# Autodesk Inventor assembly: manifold
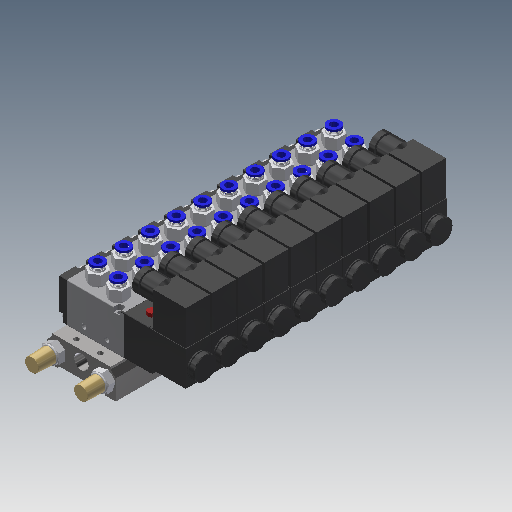
[picture p0: Inventor's stored thumbnail of the model, 512x512]
Saved by Autodesk Inventor 2017 (Build 210142000, 142)
## iProperties
Created: 2018-06-21
Part Number: manifold
Document SubType Name: Assembly
Designer: Luiz Gustavo
Author: Luiz Gustavo
## Documents named in this file (5)
- C:\Users\Luiz Gustavo\Documents\Inventor\piano-robot\manifold.iam
- C:\Users\Luiz Gustavo\Documents\Inventor\piano-robot\manifold-block.ipt
- C:\Users\Luiz Gustavo\Documents\Inventor\piano-robot\grabcad\AIRTAC 4V21008\4V21008.ipt
- C:\Users\Luiz Gustavo\Documents\Inventor\piano-robot\grabcad\AIRTAC 4V21008\BSL02.ipt
- C:\Users\Luiz Gustavo\Documents\Inventor\piano-robot\grabcad\AIRTAC 4V21008\PC602.ipt
## Components (35 placed, 4 different names)
1. manifold-block:1 — Flush:1, Flush:2, Flush:3, Rigid:1, Rigid:2, Rigid:3, Rigid:4, Rigid:5
2. BSL02:1 — Rigid:2
3. BSL02:2 — Rigid:3
4. BSL02:3 — Rigid:5
5. BSL02:4 — Rigid:4
6. 4V21008:1 — Rigid:1, Rigid:6, Rigid:7
7. 4V21008:2
8. 4V21008:3
9. 4V21008:4
10. 4V21008:5
11. 4V21008:6
12. 4V21008:7
13. 4V21008:8
14. 4V21008:9
15. 4V21008:10
16. PC602:2 — Rigid:7
17. PC602:3
18. PC602:4
19. PC602:5
20. PC602:6
21. PC602:7
22. PC602:8
23. PC602:9
24. PC602:10
25. PC602:11
26. PC602:1 — Rigid:6
27. PC602:12
28. PC602:13
29. PC602:14
30. PC602:15
31. PC602:16
32. PC602:17
33. PC602:18
34. PC602:19
35. PC602:20
## Component patterns: (10 elements, first: 4V21008:1), (10 elements, first: PC602:2), (10 elements, first: PC602:1)
## Relationships (10: WeldJoint 7, Flush 3)
- Flush:1: manifold-block:1
- Flush:2: manifold-block:1
- Flush:3: manifold-block:1
- Rigid:1 [WeldJoint]: manifold-block:1 ↔ 4V21008:1
- Rigid:2 [WeldJoint]: manifold-block:1 ↔ BSL02:1
- Rigid:3 [WeldJoint]: manifold-block:1 ↔ BSL02:2
- Rigid:4 [WeldJoint]: manifold-block:1 ↔ BSL02:4
- Rigid:5 [WeldJoint]: manifold-block:1 ↔ BSL02:3
- Rigid:6 [WeldJoint] (1 mm): 4V21008:1 ↔ PC602:1
- Rigid:7 [WeldJoint] (1 mm): 4V21008:1 ↔ PC602:2
